# Autodesk Inventor assembly: test-model-1
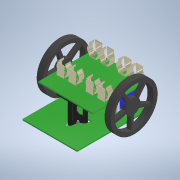
[picture p0: Inventor's stored thumbnail of the model, 180x180]
Saved by Autodesk Inventor 2022 (Build 260153000, 153)
## iProperties
Created: 2024-05-30
Part Number: test-model-1
Document SubType Name: Assembly
Designer: yamashita1
Author: yamashita1
## Documents named in this file (9)
- G:\マイドライブ\project\micro-mouse\3D-Model\test-model-1.iam
- G:\マイドライブ\project\micro-mouse\3D-Model\PCB-Bottom.ipt
- G:\マイドライブ\project\micro-mouse\3D-Model\FS90R.ipt
- G:\マイドライブ\project\micro-mouse\3D-Model\FS90R-W.ipt
- G:\マイドライブ\project\micro-mouse\3D-Model\BallCaster-H35.ipt
- G:\マイドライブ\project\micro-mouse\3D-Model\PCB-main.ipt
- G:\マイドライブ\project\micro-mouse\3D-Model\FS90-Mount2.ipt
- G:\マイドライブ\project\micro-mouse\3D-Model\FS90-Mount2-Mirror.ipt
- G:\マイドライブ\project\micro-mouse\3D-Model\AA-Cell-x2.iam
## Components (11 placed, 8 different names)
1. PCB-Bottom:1 — フラッシュ:1, フラッシュ:2, フラッシュ:3, フラッシュ:4, メイト:8, メイト:9, フラッシュ:5, メイト:10, フラッシュ:6, フラッシュ:7, メイト:13, メイト:14, メイト:16, メイト:18, メイト:19
2. FS90R:1 — フラッシュ:1, フラッシュ:2, 回転:1, メイト:8, フラッシュ:8, メイト:15
3. FS90R:2 — フラッシュ:3, フラッシュ:4, 回転:2, メイト:10, フラッシュ:9, メイト:17
4. FS90R-W:1 — 回転:1
5. FS90R-W:2 — 回転:2
6. BallCaster-H35:1 — メイト:9, フラッシュ:5
7. PCB-main:1 — フラッシュ:6, フラッシュ:7, メイト:13
8. FS90-Mount2:1 — フラッシュ:8, メイト:14, メイト:15
9. FS90-Mount2-Mirror:1 — フラッシュ:9, メイト:16, メイト:17
10. AA-Cell-x2:1 [sub-assembly] — メイト:18
11. AA-Cell-x2:2 [sub-assembly] — メイト:19
## Relationships (21: Mate 10, Flush 9, RevoluteJoint 2)
- フラッシュ:1 [Flush]: PCB-Bottom:1 ↔ FS90R:1
- フラッシュ:2 [Flush] (8 mm): PCB-Bottom:1 ↔ FS90R:1
- フラッシュ:3 [Flush]: PCB-Bottom:1 ↔ FS90R:2
- フラッシュ:4 [Flush] (-8 mm): PCB-Bottom:1 ↔ FS90R:2
- 回転:1 [RevoluteJoint]: FS90R:1 ↔ FS90R-W:1
- 回転:2 [RevoluteJoint]: FS90R:2 ↔ FS90R-W:2
- メイト:8 [Mate]: PCB-Bottom:1 ↔ FS90R:1
- メイト:9 [Mate]: PCB-Bottom:1 ↔ BallCaster-H35:1
- フラッシュ:5 [Flush]: PCB-Bottom:1 ↔ BallCaster-H35:1
- メイト:10 [Mate]: PCB-Bottom:1 ↔ FS90R:2
- フラッシュ:6 [Flush]: PCB-Bottom:1 ↔ PCB-main:1
- フラッシュ:7 [Flush]: PCB-Bottom:1 ↔ PCB-main:1
- メイト:13 [Mate] (30 mm): PCB-Bottom:1 ↔ PCB-main:1
- フラッシュ:8 [Flush]: FS90R:1 ↔ FS90-Mount2:1
- メイト:14 [Mate]: PCB-Bottom:1 ↔ FS90-Mount2:1
- メイト:15 [Mate] (0.2 mm): FS90R:1 ↔ FS90-Mount2:1
- フラッシュ:9 [Flush]: FS90R:2 ↔ FS90-Mount2-Mirror:1
- メイト:16 [Mate]: PCB-Bottom:1 ↔ FS90-Mount2-Mirror:1
- メイト:17 [Mate] (0.2 mm): FS90R:2 ↔ FS90-Mount2-Mirror:1
- メイト:18 [Mate]: PCB-Bottom:1 ↔ AA-Cell-x2:1
- メイト:19 [Mate]: PCB-Bottom:1 ↔ AA-Cell-x2:2
